# Autodesk Inventor assembly: 3_finger_gripper
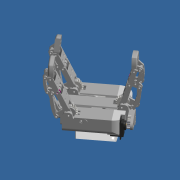
[picture p0: Inventor's stored thumbnail of the model, 180x180]
Saved by Autodesk Inventor 2016 (Build 200138000, 138)
## iProperties
Created: 2015-01-03
Part Number: 3_finger_gripper
Document SubType Name: Assembly
Designer: 4ndreas
Author: 4ndreas
## Documents named in this file (8)
- C:\Users\4ndreas\Documents\Inventor\Gripper\openHand\3_finger_gripper.iam
- C:\Users\4ndreas\Documents\Inventor\Gripper\3-Finger Gripper\Finger_clean.iam
- C:\Users\4ndreas\Documents\Inventor\Gripper\3-Finger Gripper\Finger_L.iam
- C:\Users\4ndreas\Documents\Inventor\Gripper\3-Finger Gripper\Finger_L1.iam
- C:\Users\4ndreas\Documents\Inventor\Gripper\3-Finger Gripper\kipprad.ipt
- C:\Users\4ndreas\Documents\Inventor\Gripper\3-Finger Gripper\3_finger_gripper\Konstruktions-Assistent\Stirnzahnrad13.ipt
- C:\Users\4ndreas\Documents\Inventor\Gripper\3-Finger Gripper\Gripper_coupling.ipt
- C:\Users\4ndreas\Documents\Inventor\RobotARM v2\v3\Gripper_Coupling.ipt
## Components (7 placed, 7 different names)
1. Finger_clean:1 [sub-assembly] — Passend:28, Passend:69, Passend:72, Passend:73, Passend:78, Passend:79, Passend:83, Winkel:2, Passend:87, Passend:88
2. Finger_L:1 [sub-assembly] — Passend:75, Fluchtend:1, Fluchtend:3, Drehung:1, Winkel:2, Passend:84, Passend:85
3. Finger_L1:1 [sub-assembly] — Passend:28, Passend:74, Fluchtend:1, Fluchtend:3, Drehung:1
4. kipprad:1 — Passend:82, Passend:83
5. Stirnzahnrad1:1 — Passend:84, Passend:85
6. Gripper_coupling:1 — Passend:86, Passend:87, Passend:88, Fluchtend:4, Passend:89, Passend:90
7. Gripper_Coupling:1 — Fluchtend:4, Passend:89, Passend:90
## Relationships (27: Mate 22, Flush 3, RelateRotation 1, Angle 1)
- Passend:28 [Mate]: Finger_clean:1 ↔ Finger_L1:1
- Passend:69 [Mate]: Finger_clean:1
- Passend:71 [Mate]
- Passend:72 [Mate]: Finger_clean:1
- Passend:73 [Mate]: Finger_clean:1
- Passend:74 [Mate]: Finger_L1:1
- Passend:75 [Mate]: Finger_L:1
- Passend:76 [Mate]
- Passend:77 [Mate]
- Passend:78 [Mate]: Finger_clean:1
- Passend:79 [Mate]: Finger_clean:1
- Passend:80 [Mate]
- Passend:81 [Mate]
- Fluchtend:1 [Flush]: Finger_L:1 ↔ Finger_L1:1
- Passend:82 [Mate]: kipprad:1
- Passend:83 [Mate]: Finger_clean:1 ↔ kipprad:1
- Fluchtend:3 [Flush]: Finger_L:1 ↔ Finger_L1:1
- Drehung:1 [RelateRotation] (1 ul): Finger_L:1 ↔ Finger_L1:1
- Winkel:2 [Angle] (145 deg): Finger_clean:1 ↔ Finger_L:1
- Passend:84 [Mate]: Finger_L:1 ↔ Stirnzahnrad1:1
- Passend:85 [Mate] (1 mm): Finger_L:1 ↔ Stirnzahnrad1:1
- Passend:86 [Mate]: Gripper_coupling:1
- Passend:87 [Mate]: Finger_clean:1 ↔ Gripper_coupling:1
- Passend:88 [Mate]: Finger_clean:1 ↔ Gripper_coupling:1
- Fluchtend:4 [Flush]: Gripper_coupling:1 ↔ Gripper_Coupling:1
- Passend:89 [Mate]: Gripper_coupling:1 ↔ Gripper_Coupling:1
- Passend:90 [Mate]: Gripper_coupling:1 ↔ Gripper_Coupling:1
